# Autodesk Inventor assembly: cylinder_assembly
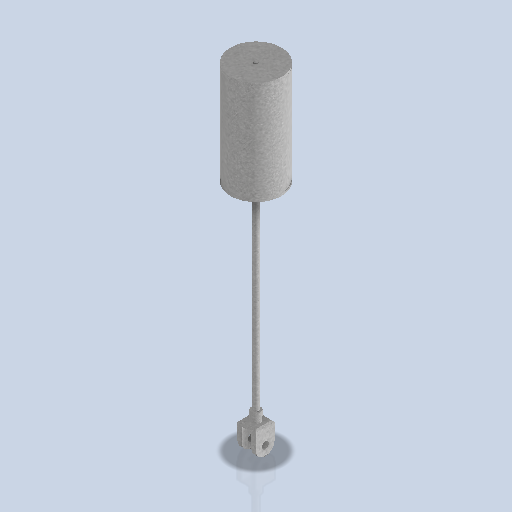
[picture p0: Inventor's stored thumbnail of the model, 512x512]
Saved by Autodesk Inventor 2024.2 (Build 282272000, 272)
## iProperties
Created: 2024-05-05
Part Number: cylinder_assembly
Document SubType Name: Assembly
Designer: Fabri
Author: Fabri
## Documents named in this file (5)
- C:\Users\Fabri\Documents\Inventor\stirlingEngine\cylinder_assembly.iam
- C:\Users\Fabri\Documents\Inventor\stirlingEngine\cylinder.ipt
- C:\Users\Fabri\Documents\Inventor\stirlingEngine\cylinder_cover_top.ipt
- C:\Users\Fabri\Documents\Inventor\stirlingEngine\welle.ipt
- C:\Users\Fabri\Documents\Inventor\stirlingEngine\top_cylinder.ipt
## Components (5 placed, 4 different names)
1. cylinder:1 — Passend:1, Einfügen:1, Einfügen:2
2. cylinder_cover_top:1 — Passend:1, Einfügen:1
3. cylinder_cover_top:2 — Einfügen:2, Passend:2
4. welle:1 — Passend:2, Passend:3, Einfügen:4
5. top_cylinder:1 — Passend:3, Einfügen:4
## Relationships (6: Mate 3, Insert 3)
- Passend:1 [Mate]: cylinder:1 ↔ cylinder_cover_top:1
- Einfügen:1 [Insert] (-3 mm): cylinder:1 ↔ cylinder_cover_top:1
- Einfügen:2 [Insert] (-3 mm): cylinder:1 ↔ cylinder_cover_top:2
- Passend:2 [Mate]: cylinder_cover_top:2 ↔ welle:1
- Passend:3 [Mate]: welle:1 ↔ top_cylinder:1
- Einfügen:4 [Insert] (-18 mm): welle:1 ↔ top_cylinder:1
